# Autodesk Inventor assembly: Assembly_Matchboxscope_injectionmolded_holo
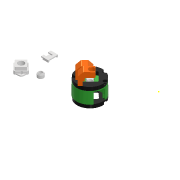
[picture p0: Inventor's stored thumbnail of the model, 180x180]
Saved by Autodesk Inventor 2022 (Build 260153000, 153)
## iProperties
Created: 2023-04-12
Part Number: Assembly_Matchboxscope_injectionmolded_holo
Document SubType Name: Assembly
Designer: diederichbenedict
Author: diederichbenedict
## Documents named in this file (11)
- C:\Users\diederichbenedict\Dropbox\Dokumente\Promotion\PROJECTS\Matchboxscope\INVENTOR\RELEASE\InjectionMolded\Assembly_Matchboxscope_injectionmolded_holo.iam
- C:\Users\diederichbenedict\Dropbox\Dokumente\Promotion\PROJECTS\Matchboxscope\INVENTOR\RELEASE\InjectionMolded\IM_Matchboxscope_base.ipt
- C:\Users\diederichbenedict\Dropbox\Dokumente\Promotion\PROJECTS\Matchboxscope\INVENTOR\RELEASE\InjectionMolded\IM_Matchboxscope_plate.ipt
- C:\Users\diederichbenedict\Dropbox\Dokumente\Promotion\PROJECTS\Matchboxscope\INVENTOR\RELEASE\InjectionMolded\IM_Lensholder.ipt
- C:\Users\diederichbenedict\Dropbox\Dokumente\Promotion\PROJECTS\Matchboxscope\INVENTOR\RELEASE\InjectionMolded\IM_Periscope.ipt
- C:\Users\diederichbenedict\Dropbox\Dokumente\Promotion\PROJECTS\Matchboxscope\INVENTOR\RELEASE\InjectionMolded\IM_ledholder.ipt
- C:\Users\diederichbenedict\Dropbox\Dokumente\Promotion\PROJECTS\Matchboxscope\INVENTOR\RELEASE\InjectionMolded\Anglerfish_Cameraspacer.ipt
- C:\Users\diederichbenedict\Dropbox\Dokumente\Promotion\PROJECTS\Matchboxscope\INVENTOR\RELEASE\InjectionMolded\00_CCTV_M12_VCM_large.ipt
- C:\Users\diederichbenedict\Dropbox\Dokumente\Promotion\PROJECTS\Matchboxscope\INVENTOR\RELEASE\InjectionMolded\IM_Lensholder_M12.ipt
- C:\Users\diederichbenedict\Dropbox\Dokumente\Promotion\PROJECTS\Matchboxscope\INVENTOR\RELEASE\InjectionMolded\Matchboxscope_M12_Lensadapter_v0.ipt
- C:\Users\diederichbenedict\Dropbox\Dokumente\Promotion\PROJECTS\Matchboxscope\INVENTOR\RELEASE\InjectionMolded\00_Turningscrew.ipt
## Components (11 placed, 10 different names)
1. IM_Matchboxscope_base:1 — Fluchtend:1
2. IM_Matchboxscope_plate:1
3. IM_Matchboxscope_plate:2 — Einfügen:4, Winkel:1
4. IM_Lensholder:1 — Fluchtend:1
5. IM_Periscope:1 — Einfügen:4, Winkel:1
6. IM_ledholder:1
7. Anglerfish_Cameraspacer:1
8. 00_CCTV_M12_VCM_large:1 — Passend:2, Winkel:2
9. IM_Lensholder_M12:1 — Passend:2, Winkel:2
10. Matchboxscope_M12_Lensadapter_v0:1
11. 00_Turningscrew:1
## Relationships (9: Insert 4, Mate 2, Angle 2, Flush 1)
- [Insert]: IM_Matchboxscope_base:1 ↔ IM_Matchboxscope_plate:1
- [Insert]: IM_Matchboxscope_base:1 ↔ IM_Matchboxscope_plate:1
- [Insert]: IM_Matchboxscope_base:1 ↔ IM_Matchboxscope_plate:2
- [Mate]: IM_Matchboxscope_base:1 ↔ IM_Matchboxscope_plate:2
- Fluchtend:1 [Flush]: IM_Matchboxscope_base:1 ↔ IM_Lensholder:1
- Einfügen:4 [Insert]: IM_Matchboxscope_plate:2 ↔ IM_Periscope:1
- Winkel:1 [Angle] (0 deg): IM_Matchboxscope_plate:2 ↔ IM_Periscope:1
- Passend:2 [Mate]: 00_CCTV_M12_VCM_large:1 ↔ IM_Lensholder_M12:1
- Winkel:2 [Angle] (45 deg): 00_CCTV_M12_VCM_large:1 ↔ IM_Lensholder_M12:1
